# Autodesk Inventor assembly: 2020-2040_left
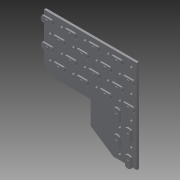
[picture p0: Inventor's stored thumbnail of the model, 180x180]
Saved by Autodesk Inventor 2014 (Build 180170000, 170)
## iProperties
Created: 2014-10-05
Part Number: 2020-2040_left
Document SubType Name: Assembly
Designer: Matthew
Author: Matthew
## Documents named in this file (3)
- C:\Users\Matthew\Documents\GitHub\CNC Mill\8020\2020-2040_left.iam
- C:\Users\Matthew\Documents\GitHub\CNC Mill\8020\2020-2040_mounting_plate.ipt
- C:\Users\Matthew\Documents\GitHub\CNC Mill\8020\0.5in_tnut.iam
## Components (21 placed, 2 different names)
1. 2020-2040_mounting_plate:1 — Insert:1, Insert:2, Insert:3, Insert:4, Insert:5, Insert:6, Insert:7, Insert:8, Insert:9, Insert:10, Insert:11, Insert:12, Insert:13, Insert:14, Insert:15, Insert:16, Insert:17, Insert:18, Insert:19, Insert:20
2. 0.5in_tnut:1 [sub-assembly] — Flush:15, Flush:16, Insert:2
3. 0.5in_tnut:2 [sub-assembly] — Flush:4, Flush:5, Flush:7, Insert:14
4. 0.5in_tnut:3 [sub-assembly] — Flush:9, Flush:10, Insert:11
5. 0.5in_tnut:4 [sub-assembly] — Flush:12, Flush:13, Insert:6
6. 0.5in_tnut:5 [sub-assembly] — Flush:5, Flush:7, Insert:13
7. 0.5in_tnut:6 [sub-assembly] — Flush:10, Insert:12
8. 0.5in_tnut:7 [sub-assembly] — Flush:11, Insert:8
9. 0.5in_tnut:8 [sub-assembly] — Flush:2, Insert:17
10. 0.5in_tnut:9 [sub-assembly] — Flush:11, Flush:12, Insert:7
11. 0.5in_tnut:10 [sub-assembly] — Flush:14, Insert:5
12. 0.5in_tnut:11 [sub-assembly] — Flush:13, Insert:3
13. 0.5in_tnut:12 [sub-assembly] — Flush:8, Insert:10
14. 0.5in_tnut:13 [sub-assembly] — Flush:16, Insert:1
15. 0.5in_tnut:14 [sub-assembly] — Flush:8, Flush:9, Insert:9
16. 0.5in_tnut:15 [sub-assembly] — Flush:14, Flush:15, Insert:4
17. 0.5in_tnut:16 [sub-assembly] — Flush:6, Insert:16
18. 0.5in_tnut:17 [sub-assembly] — Flush:4, Flush:6, Insert:15
19. 0.5in_tnut:18 [sub-assembly] — Flush:3, Insert:20
20. 0.5in_tnut:19 [sub-assembly] — Flush:3, Insert:19
21. 0.5in_tnut:20 [sub-assembly] — Flush:2, Insert:18
## Relationships (35: Insert 20, Flush 15)
- Flush:2: 0.5in_tnut:8 ↔ 0.5in_tnut:20
- Flush:3: 0.5in_tnut:18 ↔ 0.5in_tnut:19
- Flush:4: 0.5in_tnut:2 ↔ 0.5in_tnut:17
- Flush:5: 0.5in_tnut:2 ↔ 0.5in_tnut:5
- Flush:6: 0.5in_tnut:16 ↔ 0.5in_tnut:17
- Flush:7: 0.5in_tnut:2 ↔ 0.5in_tnut:5
- Flush:8: 0.5in_tnut:12 ↔ 0.5in_tnut:14
- Flush:9: 0.5in_tnut:3 ↔ 0.5in_tnut:14
- Flush:10: 0.5in_tnut:3 ↔ 0.5in_tnut:6
- Flush:11: 0.5in_tnut:7 ↔ 0.5in_tnut:9
- Flush:12: 0.5in_tnut:4 ↔ 0.5in_tnut:9
- Flush:13: 0.5in_tnut:4 ↔ 0.5in_tnut:11
- Flush:14: 0.5in_tnut:10 ↔ 0.5in_tnut:15
- Flush:15: 0.5in_tnut:1 ↔ 0.5in_tnut:15
- Flush:16: 0.5in_tnut:1 ↔ 0.5in_tnut:13
- Insert:1: 2020-2040_mounting_plate:1 ↔ 0.5in_tnut:13
- Insert:2: 2020-2040_mounting_plate:1 ↔ 0.5in_tnut:1
- Insert:3: 2020-2040_mounting_plate:1 ↔ 0.5in_tnut:11
- Insert:4: 2020-2040_mounting_plate:1 ↔ 0.5in_tnut:15
- Insert:5: 2020-2040_mounting_plate:1 ↔ 0.5in_tnut:10
- Insert:6: 2020-2040_mounting_plate:1 ↔ 0.5in_tnut:4
- Insert:7: 2020-2040_mounting_plate:1 ↔ 0.5in_tnut:9
- Insert:8: 2020-2040_mounting_plate:1 ↔ 0.5in_tnut:7
- Insert:9: 2020-2040_mounting_plate:1 ↔ 0.5in_tnut:14
- Insert:10: 2020-2040_mounting_plate:1 ↔ 0.5in_tnut:12
- Insert:11: 2020-2040_mounting_plate:1 ↔ 0.5in_tnut:3
- Insert:12: 2020-2040_mounting_plate:1 ↔ 0.5in_tnut:6
- Insert:13: 2020-2040_mounting_plate:1 ↔ 0.5in_tnut:5
- Insert:14: 2020-2040_mounting_plate:1 ↔ 0.5in_tnut:2
- Insert:15: 2020-2040_mounting_plate:1 ↔ 0.5in_tnut:17
- Insert:16: 2020-2040_mounting_plate:1 ↔ 0.5in_tnut:16
- Insert:17: 2020-2040_mounting_plate:1 ↔ 0.5in_tnut:8
- Insert:18: 2020-2040_mounting_plate:1 ↔ 0.5in_tnut:20
- Insert:19: 2020-2040_mounting_plate:1 ↔ 0.5in_tnut:19
- Insert:20: 2020-2040_mounting_plate:1 ↔ 0.5in_tnut:18
